# Autodesk Inventor assembly: intake_gearbox_outer
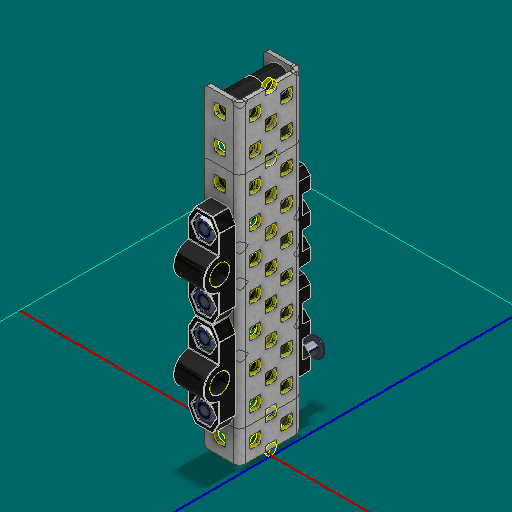
[picture p0: Inventor's stored thumbnail of the model, 512x512]
Saved by Autodesk Inventor 2025 (Build 290162000, 162)
## iProperties
Created: 2024-08-19
Part Number: intake_gearbox_outer
Document SubType Name: Assembly
Designer: averey
Author: averey
## Documents named in this file (14)
- C:\Users\avere\vex_robotics_high_stakes\hardware\cad\ATLAS\tower\structure\intake_gearbox_outer.iam
- C:\Users\avere\vex_robotics_high_stakes\hardware\cad\VEX-CAD-Inventor\Structure\C Channel\Aluminum 1x2x1\Alu C 1x2x1x8.ipt
- C:\Users\avere\vex_robotics_high_stakes\hardware\cad\VEX-CAD-Inventor\Motion\Shaft HS\HS Pillow Bearing Block.ipt
- C:\Users\avere\vex_robotics_high_stakes\hardware\cad\VEX-CAD-Inventor\Motion\Spacers\Spacer Nylon .375 OD\NSpacer .375 OD x .375.ipt
- C:\Users\avere\vex_robotics_high_stakes\hardware\cad\VEX-CAD-Inventor\Motion\Spacers\Spacer Nylon .375 OD.ipt
- C:\Users\avere\vex_robotics_high_stakes\hardware\cad\VEX-CAD-Inventor\Motion\Spacers\Spacer Nylon .375 OD\NSpacer .375 OD x .500.ipt
- C:\Users\avere\vex_robotics_high_stakes\hardware\cad\VEX-CAD-Inventor\Motion\Shaft LS\Bearing Flat.ipt
- C:\Users\avere\vex_robotics_high_stakes\hardware\cad\VEX-CAD-Inventor\Structure\Hardware\Screw Steel - Star\SScrew Star Smooth 1.500.ipt
- C:\Users\avere\vex_robotics_high_stakes\hardware\cad\VEX-CAD-Inventor\Structure\Hardware\Screw Steel - Star.ipt
- C:\Users\avere\vex_robotics_high_stakes\hardware\cad\VEX-CAD-Inventor\Structure\Hardware\Nut Thin Nylock.ipt
- C:\Users\avere\vex_robotics_high_stakes\hardware\cad\VEX-CAD-Inventor\Structure\C Channel\Aluminum 1x2x1\Alu C 1x2x1x10.ipt
- C:\Users\avere\vex_robotics_high_stakes\hardware\cad\VEX-CAD-Inventor\Motion\Shaft HS\HS Bearing Flat.ipt
- C:\Users\avere\vex_robotics_high_stakes\hardware\cad\VEX-CAD-Inventor\Structure\C Channel\Aluminum 1x2x1\Alu C 1x2x1x9.ipt
- C:\Users\avere\vex_robotics_high_stakes\hardware\cad\VEX-CAD-Inventor\Structure\Hardware\Screw Steel - Star\SScrew Star Smooth 1.750.ipt
## Components (28 placed, 11 different names)
1. Alu C 1x2x1x8:1 — Insert:32, Mate:4, Insert:33, Mate:5, Insert:34, Mate:6
2. HS Pillow Bearing Block:2 — Insert:18, Insert:20
3. NSpacer .375 OD x .375:5 — Insert:18
4. NSpacer .375 OD x .500:6 — Insert:17, Insert:33
5. NSpacer .375 OD x .375:7 — Insert:20
6. NSpacer .375 OD x .500:8 — Insert:19, Mate:5
7. Bearing Flat:2 — Insert:17, Insert:19
8. SScrew Star Smooth 1.500:3
9. SScrew Star Smooth 1.500:4
10. Nut Thin Nylock:3
11. Nut Thin Nylock:4
12. HS Pillow Bearing Block:3
13. NSpacer .375 OD x .375:9 — Insert:40
14. NSpacer .375 OD x .500:10 — Mate:4
15. NSpacer .375 OD x .375:11
16. NSpacer .375 OD x .500:12 — Insert:32
17. Bearing Flat:3 — Mate:8, Insert:41
18. SScrew Star Smooth 1.500:6
19. Nut Thin Nylock:5
20. Nut Thin Nylock:6
21. Alu C 1x2x1x10:1 — Insert:34, Mate:6, Insert:35, Mate:7, Insert:38, Insert:39
22. HS Bearing Flat:1 — Insert:35, Mate:7
23. NSpacer .375 OD x .375:13
24. NSpacer .375 OD x .500:14 — Insert:39
25. NSpacer .375 OD x .375:15
26. NSpacer .375 OD x .500:16 — Insert:38
27. Alu C 1x2x1x9:1 — Insert:40, Mate:8
28. SScrew Star Smooth 1.750:7 — Insert:41
## Relationships (34: Insert 29, Mate 5)
- [Insert]: NSpacer .375 OD x .375:5 ↔ NSpacer .375 OD x .500:6
- [Insert]: NSpacer .375 OD x .375:7 ↔ NSpacer .375 OD x .500:8
- [Insert]: Bearing Flat:2 ↔ SScrew Star Smooth 1.500:4
- [Insert]: Bearing Flat:2 ↔ SScrew Star Smooth 1.500:3
- [Insert]: HS Pillow Bearing Block:2 ↔ Nut Thin Nylock:4
- [Insert]: HS Pillow Bearing Block:2 ↔ Nut Thin Nylock:3
- Insert:17 (1.5875 mm): NSpacer .375 OD x .500:6 ↔ Bearing Flat:2
- Insert:18 (1.5875 mm): HS Pillow Bearing Block:2 ↔ NSpacer .375 OD x .375:5
- Insert:19 (1.5875 mm): NSpacer .375 OD x .500:8 ↔ Bearing Flat:2
- Insert:20 (1.5875 mm): HS Pillow Bearing Block:2 ↔ NSpacer .375 OD x .375:7
- [Insert]: NSpacer .375 OD x .375:9 ↔ NSpacer .375 OD x .500:10
- [Insert]: NSpacer .375 OD x .375:11 ↔ NSpacer .375 OD x .500:12
- [Insert]: Bearing Flat:3 ↔ SScrew Star Smooth 1.500:6
- [Insert]: HS Pillow Bearing Block:3 ↔ Nut Thin Nylock:6
- [Insert]: HS Pillow Bearing Block:3 ↔ Nut Thin Nylock:5
- [Insert] (1.5875 mm): NSpacer .375 OD x .500:10 ↔ Bearing Flat:3
- [Insert] (1.5875 mm): HS Pillow Bearing Block:3 ↔ NSpacer .375 OD x .375:9
- [Insert] (1.5875 mm): NSpacer .375 OD x .500:12 ↔ Bearing Flat:3
- [Insert] (1.5875 mm): HS Pillow Bearing Block:3 ↔ NSpacer .375 OD x .375:11
- Insert:32: Alu C 1x2x1x8:1 ↔ NSpacer .375 OD x .500:12
- Mate:4: Alu C 1x2x1x8:1 ↔ NSpacer .375 OD x .500:10
- Insert:33: Alu C 1x2x1x8:1 ↔ NSpacer .375 OD x .500:6
- Mate:5: Alu C 1x2x1x8:1 ↔ NSpacer .375 OD x .500:8
- Insert:34: Alu C 1x2x1x8:1 ↔ Alu C 1x2x1x10:1
- Mate:6: Alu C 1x2x1x8:1 ↔ Alu C 1x2x1x10:1
- Insert:35: Alu C 1x2x1x10:1 ↔ HS Bearing Flat:1
- Mate:7: Alu C 1x2x1x10:1 ↔ HS Bearing Flat:1
- [Insert]: NSpacer .375 OD x .375:13 ↔ NSpacer .375 OD x .500:14
- [Insert]: NSpacer .375 OD x .375:15 ↔ NSpacer .375 OD x .500:16
- Insert:38: Alu C 1x2x1x10:1 ↔ NSpacer .375 OD x .500:16
- Insert:39: Alu C 1x2x1x10:1 ↔ NSpacer .375 OD x .500:14
- Insert:40: NSpacer .375 OD x .375:9 ↔ Alu C 1x2x1x9:1
- Mate:8: Bearing Flat:3 ↔ Alu C 1x2x1x9:1
- Insert:41 (6.35 mm): Bearing Flat:3 ↔ SScrew Star Smooth 1.750:7
## Named parameters: d6_d41 = 0 mm, d7_d43_d41 = 0 mm, d8_d55 = 0 mm, d9_d56 = 0 mm, d10_d59 = 0 mm, d11_d60 = 0 mm, d24_d6_d41 = 0 mm, d25_d7_d43_d41 = 0 mm, d26_d8_d55 = 0 mm, d28_d10_d59 = 0 mm, d29_d11_d60 = 0 mm, d30_d18 = 1.5875 mm, d31_d19 = 1.5875 mm, d32_d20 = 1.5875 mm, d33_d21 = 1.5875 mm, d43_d65 = 0 mm
